# Autodesk Inventor assembly: uchwytak
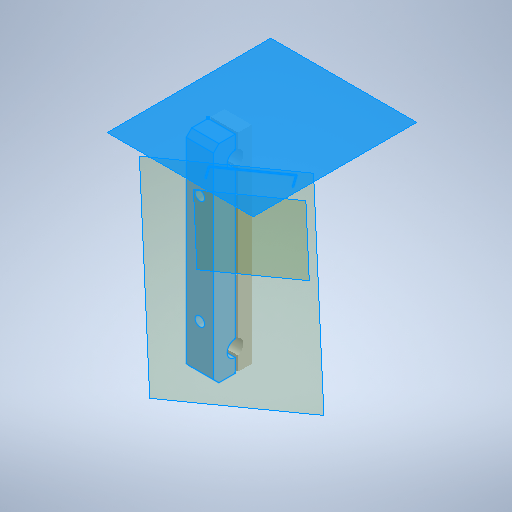
[picture p0: Inventor's stored thumbnail of the model, 512x512]
Saved by Autodesk Inventor 2025.1 (Build 291241000, 241)
## iProperties
Created: 2024-10-31
Part Number: uchwytak
Document SubType Name: Assembly
Designer: PC
Author: PC
## Documents named in this file (3)
- C:\Users\PC\Desktop\fotolito_czesci\nowe\uchwytak.iam
- C:\Users\PC\Desktop\fotolito_czesci\nowe\6_2xclamp_main.ipt
- C:\Users\PC\Desktop\fotolito_czesci\nowe\6_2xclamp_back.ipt
## Components (2 placed, 2 different names)
1. 6_2xclamp_main:1 — Równoległe:1
2. 6_2xclamp_back:1 — Równoległe:1
## Relationships (1: Flush 1)
- Równoległe:1 [Flush]: 6_2xclamp_main:1 ↔ 6_2xclamp_back:1
